# Autodesk Inventor assembly: leg2
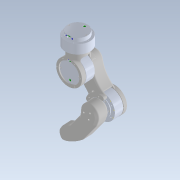
[picture p0: Inventor's stored thumbnail of the model, 180x180]
Saved by Autodesk Inventor 2020 (Build 240168000, 168)
## iProperties
Created: 2020-12-23
Part Number: leg2
Document SubType Name: Assembly
Designer: DELL
Author: DELL
## Documents named in this file (6)
- F:\SoftRobot2.0\Flexipod2.0\leg2_2020_12_22_21_58\leg2.iam
- F:\SoftRobot2.0\Flexipod2.0\RMD_X6_stator.ipt
- F:\SoftRobot2.0\Flexipod2.0\RMD_X6_rotor.ipt
- F:\SoftRobot2.0\Flexipod2.0\leg2_2020_12_22_21_58\hip_link.ipt
- F:\SoftRobot2.0\Flexipod2.0\leg2_2020_12_22_21_58\shank_link.ipt
- F:\SoftRobot2.0\Flexipod2.0\leg2_2020_12_22_21_58\thigh_link.ipt
## Components (9 placed, 5 different names)
1. RMD_X6_stator:1 — Mate:1, Flush:1, Mate:4, Mate:5
2. RMD_X6_rotor:1 — Mate:1, Flush:1, Mate:6, Mate:7, Mate:8, Mate:9
3. hip_link:1 — Mate:7, Mate:8, Mate:9, Mate:11, Mate:12, Mate:13
4. RMD_X6_stator:2 — Mate:11, Mate:12, Mate:13, Mate:15
5. RMD_X6_rotor:2 — Mate:14, Mate:20
6. thigh_link:1 — Mate:14, Mate:15, Mate:17, Mate:18, Mate:19, Mate:20
7. RMD_X6_stator:3 — Mate:17, Mate:18, Mate:19
8. RMD_X6_rotor:3 — Mate:21, Mate:22, Mate:23
9. shank_link:1 — Mate:21, Mate:22, Mate:23
## Relationships (24: Mate 21, Flush 3)
- Mate:1: RMD_X6_stator:1 ↔ RMD_X6_rotor:1
- Flush:1 (-3 mm): RMD_X6_stator:1 ↔ RMD_X6_rotor:1
- Mate:4: RMD_X6_stator:1
- Mate:5: RMD_X6_stator:1
- Mate:6: RMD_X6_rotor:1
- Mate:7: RMD_X6_rotor:1 ↔ hip_link:1
- Mate:8: RMD_X6_rotor:1 ↔ hip_link:1
- Mate:9: RMD_X6_rotor:1 ↔ hip_link:1
- [Mate]: RMD_X6_stator:2 ↔ RMD_X6_rotor:2
- [Flush] (-3 mm): RMD_X6_stator:2 ↔ RMD_X6_rotor:2
- Mate:11: hip_link:1 ↔ RMD_X6_stator:2
- Mate:12: hip_link:1 ↔ RMD_X6_stator:2
- Mate:13: hip_link:1 ↔ RMD_X6_stator:2
- Mate:14: RMD_X6_rotor:2 ↔ thigh_link:1
- Mate:15: RMD_X6_stator:2 ↔ thigh_link:1
- [Mate]: RMD_X6_stator:3 ↔ RMD_X6_rotor:3
- [Flush] (-3 mm): RMD_X6_stator:3 ↔ RMD_X6_rotor:3
- Mate:17: thigh_link:1 ↔ RMD_X6_stator:3
- Mate:18: thigh_link:1 ↔ RMD_X6_stator:3
- Mate:19: thigh_link:1 ↔ RMD_X6_stator:3
- Mate:20: RMD_X6_rotor:2 ↔ thigh_link:1
- Mate:21: RMD_X6_rotor:3 ↔ shank_link:1
- Mate:22: RMD_X6_rotor:3 ↔ shank_link:1
- Mate:23: RMD_X6_rotor:3 ↔ shank_link:1
## Named parameters: d27_d0 = 0 mm, d28_d1 = -3 mm, d34_d27_d0 = 0 mm, d35_d28_d1 = -3 mm
